# Autodesk Inventor assembly: Assembly1
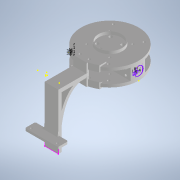
[picture p0: Inventor's stored thumbnail of the model, 180x180]
Saved by Autodesk Inventor 2021 (Build 250183000, 183)
## iProperties
Created: 2023-04-27
Part Number: Assembly1
Document SubType Name: Assembly
Designer: mahmo
Author: mahmo
## Documents named in this file (4)
- D:\AsU\semesters\senior 2\sem 2\new_gripper\send_again_to_ashraf\Assembly1.iam
- D:\AsU\semesters\senior 2\sem 2\new_gripper\manga.ipt
- D:\AsU\semesters\senior 2\sem 2\new_gripper\tool_holder.ipt
- D:\AsU\semesters\senior 2\sem 2\new_gripper\Part3.ipt
## Components (3 placed, 3 different names)
1. tool_holder:1 — Mate:1, Mate:2, Mate:3, Mate:4, Mate:7, Mate:8, Mate:9
2. Part3:1 — Mate:1, Mate:2, Mate:5, Mate:6
3. manga:1 — Mate:3, Mate:4, Mate:5, Mate:6, Mate:7, Mate:8, Mate:9
## Relationships (9: Mate 9)
- Mate:1: tool_holder:1 ↔ Part3:1
- Mate:2: tool_holder:1 ↔ Part3:1
- Mate:3: tool_holder:1 ↔ manga:1
- Mate:4: tool_holder:1 ↔ manga:1
- Mate:5: Part3:1 ↔ manga:1
- Mate:6: Part3:1 ↔ manga:1
- Mate:7: tool_holder:1 ↔ manga:1
- Mate:8: tool_holder:1 ↔ manga:1
- Mate:9: tool_holder:1 ↔ manga:1
